# Autodesk Inventor assembly: Assembly
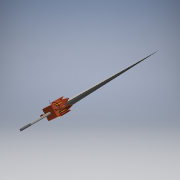
[picture p0: Inventor's stored thumbnail of the model, 180x180]
Saved by Autodesk Inventor 2017 (Build 210142000, 142)
## iProperties
Created: 2019-06-22
Part Number: Assembly
Document SubType Name: Assembly
Designer: Ole Simmering
Author: Ole Simmering
## Documents named in this file (5)
- C:\Users\Ole Simmering\Documents\3d modelling fun\Stiletto Dagger\Assembly.iam
- C:\Users\Ole Simmering\Documents\3d modelling fun\Stiletto Dagger\Blade.ipt
- C:\Users\Ole Simmering\Documents\3d modelling fun\Stiletto Dagger\TopFlower.ipt
- C:\Users\Ole Simmering\Documents\3d modelling fun\Stiletto Dagger\Spacer.ipt
- C:\Users\Ole Simmering\Documents\3d modelling fun\Stiletto Dagger\Guard.ipt
## Components (4 placed, 4 different names)
1. Blade:1 — Mate:1, Flush:1, Mate:2, Mate:3, Mate:6
2. TopFlower:1 — Mate:1, Flush:1, Angle:1
3. Spacer:1 — Mate:2, Mate:3, Mate:5
4. Guard:1 — Mate:5, Mate:6, Angle:1
## Relationships (7: Mate 5, Flush 1, Angle 1)
- Mate:1: Blade:1 ↔ TopFlower:1
- Flush:1: Blade:1 ↔ TopFlower:1
- Mate:2: Blade:1 ↔ Spacer:1
- Mate:3: Blade:1 ↔ Spacer:1
- Mate:5: Spacer:1 ↔ Guard:1
- Mate:6: Blade:1 ↔ Guard:1
- Angle:1 (0 deg): TopFlower:1 ↔ Guard:1
